# Autodesk Inventor assembly: couple extension arm motor bottom + pulleys
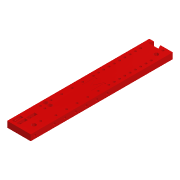
[picture p0: Inventor's stored thumbnail of the model, 180x180]
Saved by Autodesk Inventor 2020 (Build 240168000, 168)
## iProperties
Created: 2019-12-16
Part Number: couple extension arm motor bottom + pulleys
Document SubType Name: Assembly
Designer: ball
Author: ball
## Documents named in this file (3)
- C:\FTC\FTC8863CAD\2019 Robot\Delivery\extension arm\couple extension arm motor bottom + pulleys.iam
- C:\FTC\FTC8863CAD\2019 Robot\Delivery\extension arm\Coupler extension arm motor.ipt
- C:\FTC\FTC8863CAD\2019 Robot\Delivery\plastic pulley deep u.ipt
## Components (2 placed, 2 different names)
1. Coupler extension arm motor:1 — Mate:7, Mate:8
2. plastic pulley deep u:2 — Mate:7, Mate:8
## Relationships (2: Mate 2)
- Mate:7: Coupler extension arm motor:1 ↔ plastic pulley deep u:2
- Mate:8: Coupler extension arm motor:1 ↔ plastic pulley deep u:2
